# Autodesk Inventor assembly: 50_1 Stepper Gearbox
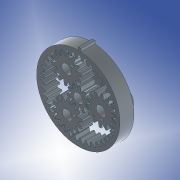
[picture p0: Inventor's stored thumbnail of the model, 180x180]
Saved by Autodesk Inventor 2017 SP1 (Build 210196100, 196)
## iProperties
Created: 2017-07-05
Part Number: 50_1 Stepper Gearbox
Document SubType Name: Assembly
Designer: Zach
Author: Zach
## Documents named in this file (8)
- C:\Users\Zach\Documents\GitHub\cr-laundry-robot\lib\50_1 Stepper Gearbox\50_1 Stepper Gearbox.iam
- C:\Users\Zach\Documents\GitHub\cr-laundry-robot\lib\50_1 Stepper Gearbox\50_1 Stepper Gearbox\Design Accelerator\Spur Gears1.iam
- C:\Users\Zach\Documents\GitHub\cr-laundry-robot\lib\50_1 Stepper Gearbox\50_1 Stepper Gearbox\Design Accelerator\Spur Gears2.iam
- C:\Users\Zach\Documents\GitHub\cr-laundry-robot\lib\50_1 Stepper Gearbox\50_1 Stepper Gearbox\Design Accelerator\Spur Gears3.iam
- C:\Users\Zach\Documents\GitHub\cr-laundry-robot\lib\50_1 Stepper Gearbox\Carrier.ipt
- C:\Users\Zach\Documents\GitHub\cr-laundry-robot\lib\50_1 Stepper Gearbox\50_1 Stepper Gearbox\Design Accelerator\Spur Gears4.iam
- C:\Users\Zach\Documents\GitHub\cr-laundry-robot\lib\50_1 Stepper Gearbox\50_1 Stepper Gearbox\Design Accelerator\Spur Gears5.iam
- C:\Users\Zach\Documents\GitHub\cr-laundry-robot\lib\50_1 Stepper Gearbox\50_1 Stepper Gearbox\Design Accelerator\Spur Gears6.iam
## Components (11 placed, 2 different names)
1. Spur Gears:1 [sub-assembly] — Flush:1, Flush:2, Flush:3, Mate:8, Mate:24, Mate:27, Mate:28, Mate:29, Mate:30
2. Spur Gears:2 [sub-assembly] — Flush:2, Mate:3, Mate:5, Mate:13, Mate:14
3. Spur Gears:3 [sub-assembly] — Flush:3, Mate:27
4. Spur Gears:4 [sub-assembly] — Flush:1, Mate:1, Mate:4, Mate:15, Mate:16
5. Spur Gears:5 [sub-assembly] — Mate:2, Mate:6, Mate:18, Mate:20
6. Carrier:1 — Mate:1, Mate:2, Mate:3, Mate:4, Mate:5, Mate:6, Mate:8, Mate:12
7. Spur Gears:6 [sub-assembly] — Mate:12, Mate:13, Mate:14, Rotation:5, Flush:4, Rotation:6
8. Spur Gears:7 [sub-assembly] — Mate:18, Mate:20, Rotation:8
9. Spur Gears:8 [sub-assembly] — Mate:15, Mate:16, Rotation:7
10. Spur Gears:9 [sub-assembly] — Rotation:5, Mate:23, Rotation:7, Rotation:8
11. Spur Gears:10 [sub-assembly] — Mate:23, Flush:4, Rotation:6
## Relationships (28: Mate 20, Flush 4, RelateRotation 4)
- Flush:1: Spur Gears:1 ↔ Spur Gears:4
- Flush:2: Spur Gears:1 ↔ Spur Gears:2
- Flush:3: Spur Gears:1 ↔ Spur Gears:3
- Mate:1: Spur Gears:4 ↔ Carrier:1
- Mate:2: Spur Gears:5 ↔ Carrier:1
- Mate:3: Spur Gears:2 ↔ Carrier:1
- Mate:4: Spur Gears:4 ↔ Carrier:1
- Mate:5: Spur Gears:2 ↔ Carrier:1
- Mate:6: Spur Gears:5 ↔ Carrier:1
- Mate:8: Spur Gears:1 ↔ Carrier:1
- Mate:12: Carrier:1 ↔ Spur Gears:6
- Mate:13: Spur Gears:2 ↔ Spur Gears:6
- Mate:14: Spur Gears:2 ↔ Spur Gears:6
- Mate:15: Spur Gears:4 ↔ Spur Gears:8
- Mate:16: Spur Gears:4 ↔ Spur Gears:8
- Mate:18: Spur Gears:5 ↔ Spur Gears:7
- Mate:20: Spur Gears:5 ↔ Spur Gears:7
- Rotation:5 [RelateRotation] (1 ul): Spur Gears:6 ↔ Spur Gears:9
- Mate:23: Spur Gears:9 ↔ Spur Gears:10
- Flush:4: Spur Gears:6 ↔ Spur Gears:10
- Rotation:6 [RelateRotation] (3 ul): Spur Gears:6 ↔ Spur Gears:10
- Rotation:7 [RelateRotation] (1 ul): Spur Gears:8 ↔ Spur Gears:9
- Rotation:8 [RelateRotation] (1 ul): Spur Gears:7 ↔ Spur Gears:9
- Mate:24: Spur Gears:1
- Mate:27: Spur Gears:1 ↔ Spur Gears:3
- Mate:28: Spur Gears:1
- Mate:29: Spur Gears:1
- Mate:30: Spur Gears:1
